# Autodesk Inventor assembly: Trilho 5 min montado
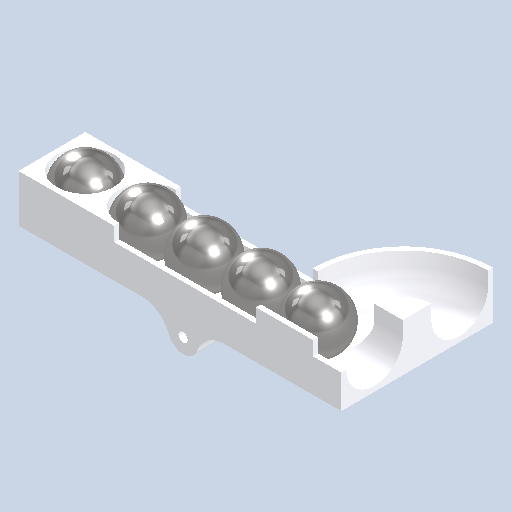
[picture p0: Inventor's stored thumbnail of the model, 512x512]
Saved by Autodesk Inventor 2024 (Build 280153000, 153)
## iProperties
Created: 2023-05-16
Part Number: Trilho 5 min montado
Document SubType Name: Assembly
Designer: jpjoa
Mass: 148.332 g
Surface Area: 166.367 cm^2
Volume: 32.2617 cm^3
Density: 4.59778 g/cm^3
Author: jpjoa
## Documents named in this file (3)
- G:\.shortcut-targets-by-id\16j0rtmAzHYi4Hd3siOhaEHA2SaTRFf-m\Marbles - Peças novas\Trilho 5 min montado.iam
- G:\.shortcut-targets-by-id\16j0rtmAzHYi4Hd3siOhaEHA2SaTRFf-m\Marbles - Peças novas\Trilho 5 min.ipt
- G:\.shortcut-targets-by-id\16j0rtmAzHYi4Hd3siOhaEHA2SaTRFf-m\Marbles - Peças novas\Bola.ipt
## Components (6 placed, 2 different names)
1. Trilho 5 min:1 — Coincidente:1, Coincidente:2, Coincidente:3, Coincidente:4, Coincidente:5
2. Bola:1 — Coincidente:1
3. Bola:2 — Coincidente:2, Tangente:1
4. Bola:3 — Coincidente:3, Tangente:2, Tangente:3
5. Bola:4 — Coincidente:4, Tangente:3
6. Bola:5 — Coincidente:5, Tangente:1, Tangente:2
## Relationships (8: Mate 5, Tangent 3)
- Coincidente:1 [Mate]: Trilho 5 min:1 ↔ Bola:1
- Coincidente:2 [Mate]: Trilho 5 min:1 ↔ Bola:2
- Coincidente:3 [Mate]: Trilho 5 min:1 ↔ Bola:3
- Coincidente:4 [Mate]: Trilho 5 min:1 ↔ Bola:4
- Coincidente:5 [Mate]: Trilho 5 min:1 ↔ Bola:5
- Tangente:1: Bola:2 ↔ Bola:5
- Tangente:2: Bola:3 ↔ Bola:5
- Tangente:3: Bola:3 ↔ Bola:4
